# Autodesk Inventor assembly: Antrieb
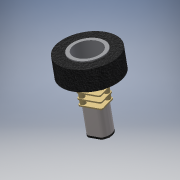
[picture p0: Inventor's stored thumbnail of the model, 180x180]
Saved by Autodesk Inventor 2017 (Build 210142000, 142)
## iProperties
Part Number: Antrieb
Material: Generisch
Document SubType Name: Assembly
Designer: Enno-LT
Author: Enno-LT
## Documents named in this file (4)
- C:\Users\Enno\Desktop\Kugelprojekt\CAD\Antrieb.iam
- C:\Users\Enno\Desktop\Kugelprojekt\CAD\Antriebsrad_V1.ipt
- C:\Users\Enno\Documents\Inventor\Content Center Files\R2017\de-DE\AS 1427(10)\AS 1427 - M2 x 5(7).ipt
- C:\Users\Enno\Desktop\Kugelprojekt\CAD\SPG10 Motor.ipt
## Components (3 placed, 3 different names)
1. Antriebsrad_V1:1 — Passend:2, Fluchtend:1, Passend:4
2. SPG10 Motor:1 — Passend:2, Fluchtend:1, Passend:5
3. AS 1427 (8) - Metrisch M2 x 5:2 — Passend:4, Passend:5
## Relationships (4: Mate 3, Flush 1)
- Passend:2 [Mate]: Antriebsrad_V1:1 ↔ SPG10 Motor:1
- Fluchtend:1 [Flush]: Antriebsrad_V1:1 ↔ SPG10 Motor:1
- Passend:4 [Mate]: Antriebsrad_V1:1 ↔ AS 1427 (8) - Metrisch M2 x 5:2
- Passend:5 [Mate]: SPG10 Motor:1 ↔ AS 1427 (8) - Metrisch M2 x 5:2
